# Autodesk Inventor assembly: SHD-25-xxx-2SH
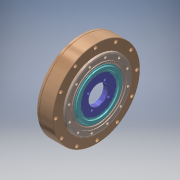
[picture p0: Inventor's stored thumbnail of the model, 180x180]
Saved by Autodesk Inventor 2018 (Build 220112000, 112)
## iProperties
Created: 2020-07-02
Part Number: SHD-25-xxx-2SH
Material: 一般
Document SubType Name: Assembly
Designer: wk415
Author: wk415
## Documents named in this file (6)
- C:\Users\wk415\Google Drive (wk415937@gmail.com)\01-Projects\[NFU] I.R.S. Lab\L.A.E.P.K. (Independent Study)\1-Projects\LAEPK-3d-model\Inventor\機械\HarmonicDrive\SHD-25-xxx-2SH.iam
- C:\Users\wk415\Google Drive (wk415937@gmail.com)\01-Projects\[NFU] I.R.S. Lab\L.A.E.P.K. (Independent Study)\1-Projects\LAEPK-3d-model\Inventor\機械\HarmonicDrive\SHD-25-2SH-CS.ipt
- C:\Users\wk415\Google Drive (wk415937@gmail.com)\01-Projects\[NFU] I.R.S. Lab\L.A.E.P.K. (Independent Study)\1-Projects\LAEPK-3d-model\Inventor\機械\HarmonicDrive\SHD-25-2SH-FS2.ipt
- C:\Users\wk415\Google Drive (wk415937@gmail.com)\01-Projects\[NFU] I.R.S. Lab\L.A.E.P.K. (Independent Study)\1-Projects\LAEPK-3d-model\Inventor\機械\HarmonicDrive\SHD-25-2SH-FS.ipt
- C:\Users\wk415\Google Drive (wk415937@gmail.com)\01-Projects\[NFU] I.R.S. Lab\L.A.E.P.K. (Independent Study)\1-Projects\LAEPK-3d-model\Inventor\機械\HarmonicDrive\25 WG BEARING DS.ipt
- C:\Users\wk415\Google Drive (wk415937@gmail.com)\01-Projects\[NFU] I.R.S. Lab\L.A.E.P.K. (Independent Study)\1-Projects\LAEPK-3d-model\Inventor\機械\HarmonicDrive\SHD-25-2SH-WG.ipt
## Components (5 placed, 5 different names)
1. SHD-25-2SH-CS:1 — 貼合:3, 貼合:4, 齊平:1, 齊平:2
2. SHD-25-2SH-FS2:1 — 貼合:1, 貼合:2, 貼合:3, 貼合:6, 齊平:1
3. SHD-25-2SH-FS:1 — 貼合:1, 貼合:2, 貼合:6
4. 25 WG BEARING DS:1 — 貼合:4, 貼合:5, 齊平:2, 齊平:3
5. SHD-25-2SH-WG:1 — 貼合:5, 齊平:3
## Relationships (9: Mate 6, Flush 3)
- 貼合:1 [Mate]: SHD-25-2SH-FS2:1 ↔ SHD-25-2SH-FS:1
- 貼合:2 [Mate]: SHD-25-2SH-FS2:1 ↔ SHD-25-2SH-FS:1
- 貼合:3 [Mate]: SHD-25-2SH-CS:1 ↔ SHD-25-2SH-FS2:1
- 貼合:4 [Mate]: SHD-25-2SH-CS:1 ↔ 25 WG BEARING DS:1
- 貼合:5 [Mate]: 25 WG BEARING DS:1 ↔ SHD-25-2SH-WG:1
- 貼合:6 [Mate]: SHD-25-2SH-FS2:1 ↔ SHD-25-2SH-FS:1
- 齊平:1 [Flush] (2.82 mm): SHD-25-2SH-CS:1 ↔ SHD-25-2SH-FS2:1
- 齊平:2 [Flush] (0.69 mm): SHD-25-2SH-CS:1 ↔ 25 WG BEARING DS:1
- 齊平:3 [Flush]: 25 WG BEARING DS:1 ↔ SHD-25-2SH-WG:1
